# Autodesk Inventor assembly: 活塞顶杆
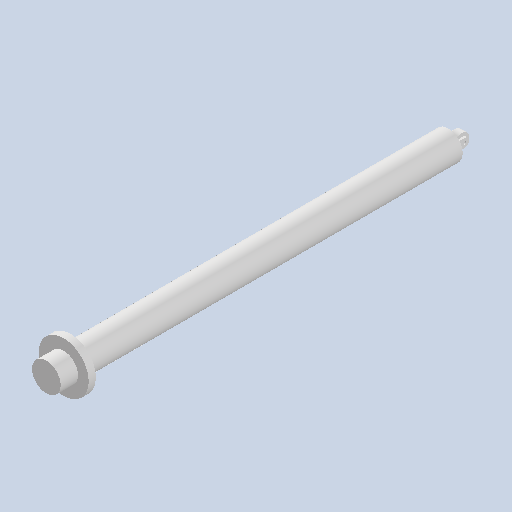
[picture p0: Inventor's stored thumbnail of the model, 512x512]
Saved by Autodesk Inventor 2022 (Build 260153000, 153)
## iProperties
Created: 2023-02-22
Part Number: 活塞顶杆
Document SubType Name: Assembly
Designer: 李承轩
Author: 李承轩
## Documents named in this file (3)
- D:\Person products\发动机模型\活塞顶杆.iam
- D:\Person products\发动机模型\顶杆.ipt
- D:\Person products\发动机模型\轮.ipt
## Components (2 placed, 2 different names)
1. 顶杆:1 — 插入:1
2. 轮:1 — 插入:1
## Relationships (1: Insert 1)
- 插入:1 [Insert] (0.5 mm): 顶杆:1 ↔ 轮:1
